# Autodesk Inventor assembly: Power Switch
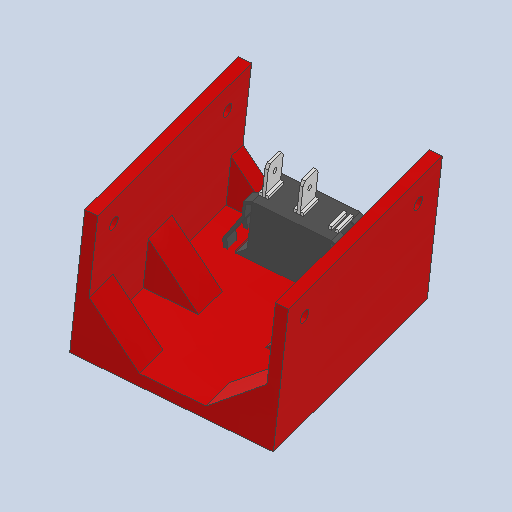
[picture p0: Inventor's stored thumbnail of the model, 512x512]
Saved by Autodesk Inventor 2022 (Build 260153000, 153)
## iProperties
Created: 2021-11-08
Part Number: Power Switch
Document SubType Name: Assembly
Designer: TakeHomePC
Author: TakeHomePC
## Documents named in this file (3)
- C:\Users\matt\Documents\Inventor\FTC\2022-23 FTC\Electronics\Power Switch.iam
- C:\Users\matt\Documents\Inventor\FTC\2022-23 FTC\Electronics\Switch power rocker.ipt
- C:\Users\matt\Documents\Inventor\FTC\2022-23 FTC\Electronics\Power Switch Shroud.ipt
## Components (2 placed, 2 different names)
1. Switch power rocker:1 — Mate:2, Mate:3, Flush:1
2. Power Switch Shroud:1 — Mate:2, Mate:3, Flush:1
## Relationships (3: Mate 2, Flush 1)
- Mate:2: Switch power rocker:1 ↔ Power Switch Shroud:1
- Mate:3 (0.5 mm): Switch power rocker:1 ↔ Power Switch Shroud:1
- Flush:1 (5.102 mm): Switch power rocker:1 ↔ Power Switch Shroud:1
